# Autodesk Inventor assembly: myCobot
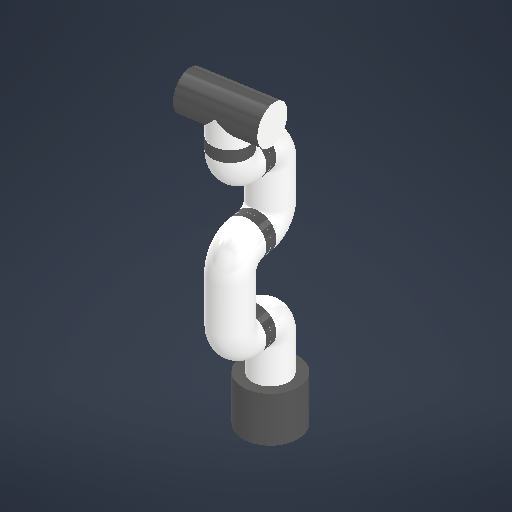
[picture p0: Inventor's stored thumbnail of the model, 512x512]
Saved by Autodesk Inventor 2026.1 (Build 301233020, 233B)
## iProperties
Created: 2025-11-06
Part Number: myCobot
Document SubType Name: Assembly
Designer: rodri
Author: rodri
## Documents named in this file (7)
- D:\Documentos\inventor\myCobot.iam
- D:\Documentos\inventor\Dron\basePlate.ipt
- D:\Documentos\inventor\Dron\lowerArm.ipt
- D:\Documentos\inventor\Dron\pitchArm.ipt
- D:\Documentos\inventor\Dron\rollArm.ipt
- D:\Documentos\inventor\Dron\upperArm.ipt
- D:\Documentos\inventor\Dron\baseArm.ipt
## Components (6 placed, 6 different names)
1. basePlate:1 — De rotación:1
2. lowerArm:1 — De rotación:2, De rotación:3
3. pitchArm:1 — De rotación:4, De rotación:5
4. rollArm:1 — De rotación:5
5. upperArm:1 — De rotación:3, De rotación:4
6. baseArm:1 — De rotación:1, De rotación:2
## Relationships (5: RevoluteJoint 5)
- De rotación:1 [RevoluteJoint]: basePlate:1 ↔ baseArm:1
- De rotación:2 [RevoluteJoint]: lowerArm:1 ↔ baseArm:1
- De rotación:3 [RevoluteJoint]: lowerArm:1 ↔ upperArm:1
- De rotación:4 [RevoluteJoint]: pitchArm:1 ↔ upperArm:1
- De rotación:5 [RevoluteJoint]: pitchArm:1 ↔ rollArm:1
